# Autodesk Inventor assembly: NewClaw
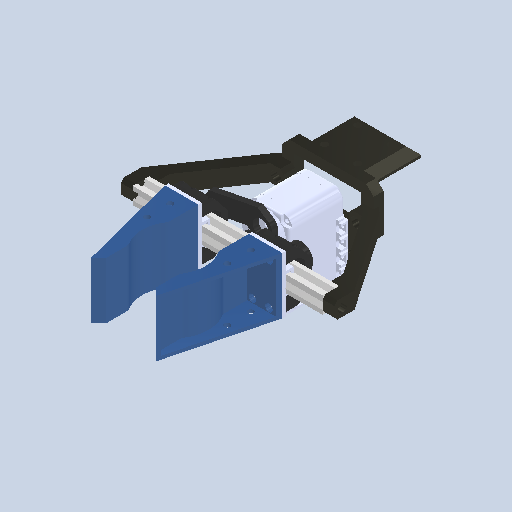
[picture p0: Inventor's stored thumbnail of the model, 512x512]
Saved by Autodesk Inventor 2024.2 (Build 282272000, 272)
## iProperties
Created: 2025-01-07
Part Number: NewClaw
Document SubType Name: Assembly
Designer: migue
Author: migue
## Documents named in this file (12)
- C:\Users\Admin\Documents\GitHub\ManipuladorCartesiano\DiseñoMecánico\Assemblies\NewClaw.iam
- C:\Users\Admin\Documents\GitHub\ManipuladorCartesiano\DiseñoMecánico\AcrylicPieces\ServoCarrier.ipt
- C:\Users\Admin\Documents\GitHub\ManipuladorCartesiano\DiseñoMecánico\Axis\AxisZ\MovingPlate\AP10x10.ipt
- C:\Users\Admin\Documents\GitHub\ManipuladorCartesiano\DiseñoMecánico\Axis\AxisZ\MovingPlate\MechanismArm.ipt
- C:\Users\Admin\Documents\GitHub\ManipuladorCartesiano\DiseñoMecánico\Motors\DynamixelAX12A\Pieces\AX12 middle.STEP.ipt
- C:\Users\Admin\Documents\GitHub\ManipuladorCartesiano\DiseñoMecánico\Motors\DynamixelAX12A\Pieces\AX12 Back.STEP.ipt
- C:\Users\Admin\Documents\GitHub\ManipuladorCartesiano\DiseñoMecánico\Motors\DynamixelAX12A\Pieces\AX12 Front.STEP.ipt
- C:\Users\Admin\Documents\GitHub\ManipuladorCartesiano\DiseñoMecánico\Motors\DynamixelAX12A\Pieces\Axel.STEP.ipt
- C:\Users\Admin\Documents\GitHub\ManipuladorCartesiano\DiseñoMecánico\Axis\AxisZ\MovingPlate\GripperSupport.ipt
- C:\Users\Admin\Documents\GitHub\ManipuladorCartesiano\DiseñoMecánico\Axis\AxisZ\MovingPlate\SliderPiece.ipt
- C:\Users\Admin\Documents\GitHub\ManipuladorCartesiano\DiseñoMecánico\Axis\AxisZ\MovingPlate\HoldingArms.ipt
- C:\Users\Admin\Documents\GitHub\ManipuladorCartesiano\DiseñoMecánico\Axis\AxisZ\Gripper.ipt
## Components (16 placed, 11 different names)
1. MechanismArm:1 — Mate:30, Mate:31, Mate:33
2. MechanismArm:2 — Mate:29, Mate:32, Mate:36
3. Axel.STEP:1 — Mate:24, Mate:25, Mate:29, Mate:30, Mate:31, Mate:32
4. GripperSupport:4 — Mate:21, Mate:22, Mate:23, Mate:36
5. GripperSupport:5 — Mate:18, Mate:19, Mate:20, Mate:33
6. SliderPiece:1 — Mate:15, Mate:16, Mate:17, Mate:21, Mate:23, Mate:37, Mate:38
7. SliderPiece:2 — Mate:9, Mate:10, Mate:11, Mate:18, Mate:19, Mate:20, Mate:34, Mate:35
8. AP10x10:1 — Mate:12, Mate:13, Mate:14, Mate:34, Mate:35, Mate:37, Mate:38
9. HoldingArms:1 — Mate:3, Mate:4, Mate:12, Mate:13
10. HoldingArms:2 — Mate:1, Mate:2, Mate:14
11. Gripper:1 — Mate:9, Mate:10, Mate:11
12. Gripper:2 — Mate:15, Mate:16, Mate:17, Mate:22
13. ServoCarrier:2 — Mate:1, Mate:2, Mate:3, Mate:4, Mate:26, Mate:27, Mate:28
14. AX12 middle.STEP:1 — Mate:5, Mate:6, Mate:7, Mate:8
15. AX12 Back.STEP:1 — Mate:5, Mate:6, Mate:26, Mate:27, Mate:28
16. AX12 Front.STEP:1 — Mate:7, Mate:8, Mate:24, Mate:25
## Relationships (38: Mate 38)
- Mate:1: HoldingArms:2 ↔ ServoCarrier:2
- Mate:2: HoldingArms:2 ↔ ServoCarrier:2
- Mate:3: HoldingArms:1 ↔ ServoCarrier:2
- Mate:4: HoldingArms:1 ↔ ServoCarrier:2
- Mate:5: AX12 middle.STEP:1 ↔ AX12 Back.STEP:1
- Mate:6: AX12 middle.STEP:1 ↔ AX12 Back.STEP:1
- Mate:7: AX12 middle.STEP:1 ↔ AX12 Front.STEP:1
- Mate:8: AX12 middle.STEP:1 ↔ AX12 Front.STEP:1
- Mate:9: SliderPiece:2 ↔ Gripper:1
- Mate:10: SliderPiece:2 ↔ Gripper:1
- Mate:11: SliderPiece:2 ↔ Gripper:1
- Mate:12: AP10x10:1 ↔ HoldingArms:1
- Mate:13: AP10x10:1 ↔ HoldingArms:1
- Mate:14: AP10x10:1 ↔ HoldingArms:2
- Mate:15: SliderPiece:1 ↔ Gripper:2
- Mate:16: SliderPiece:1 ↔ Gripper:2
- Mate:17: SliderPiece:1 ↔ Gripper:2
- Mate:18: GripperSupport:5 ↔ SliderPiece:2
- Mate:19: GripperSupport:5 ↔ SliderPiece:2
- Mate:20: GripperSupport:5 ↔ SliderPiece:2
- Mate:21: GripperSupport:4 ↔ SliderPiece:1
- Mate:22: GripperSupport:4 ↔ Gripper:2
- Mate:23: GripperSupport:4 ↔ SliderPiece:1
- Mate:24: Axel.STEP:1 ↔ AX12 Front.STEP:1
- Mate:25: Axel.STEP:1 ↔ AX12 Front.STEP:1
- Mate:26: ServoCarrier:2 ↔ AX12 Back.STEP:1
- Mate:27: ServoCarrier:2 ↔ AX12 Back.STEP:1
- Mate:28: ServoCarrier:2 ↔ AX12 Back.STEP:1
- Mate:29: MechanismArm:2 ↔ Axel.STEP:1
- Mate:30: MechanismArm:1 ↔ Axel.STEP:1
- Mate:31: MechanismArm:1 ↔ Axel.STEP:1
- Mate:32: MechanismArm:2 ↔ Axel.STEP:1
- Mate:33: MechanismArm:1 ↔ GripperSupport:5
- Mate:34: SliderPiece:2 ↔ AP10x10:1
- Mate:35: SliderPiece:2 ↔ AP10x10:1
- Mate:36: MechanismArm:2 ↔ GripperSupport:4
- Mate:37: SliderPiece:1 ↔ AP10x10:1
- Mate:38: SliderPiece:1 ↔ AP10x10:1
